# Autodesk Inventor assembly: RobotMK1
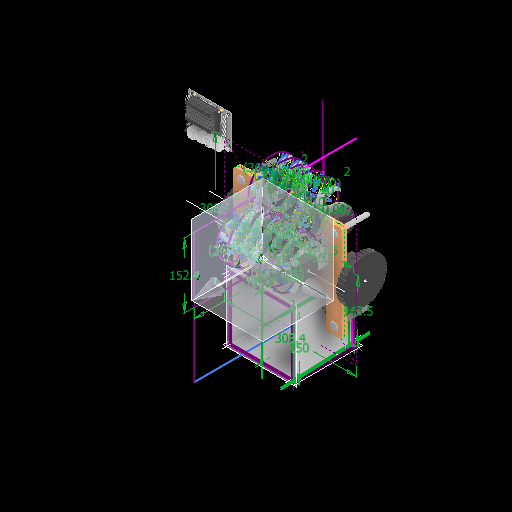
[picture p0: Inventor's stored thumbnail of the model, 512x512]
Saved by Autodesk Inventor 2025 (Build 290162000, 162)
## iProperties
Created: 2024-11-11
Part Number: RobotMK1
Document SubType Name: Assembly
Designer: Trevor
Author: Trevor
## Documents named in this file (18)
- C:\Users\Trevor\Documents\GitHub\USA-Robotic-Club-2024\assests\RobotMK1.iam
- C:\Users\Trevor\Documents\GitHub\USA-Robotic-Club-2024\assests\Newest base v1.ipt
- C:\Users\Trevor\Documents\GitHub\USA-Robotic-Club-2024\assests\17hm08-1204s-nema17-pancake-21mm-1.snapshot.2\17HM08-1204S Nema17 Pancake 21mm\17HM08-1204S Nema17 Pancake 21mm.ipt
- C:\Users\Trevor\Documents\GitHub\USA-Robotic-Club-2024\assests\Part147.ipt
- C:\Users\Trevor\Documents\GitHub\USA-Robotic-Club-2024\assests\nema-17-40mm-stepper-motor-1.snapshot.22\17HM15-0904S\17HM15-0904S\17HM15-0904S.ipt
- C:\Users\Trevor\Documents\GitHub\USA-Robotic-Club-2024\assests\RobotWheelMK1.ipt
- C:\Users\Trevor\Documents\GitHub\USA-Robotic-Club-2024\assests\Nema17WheelMotorMount.ipt
- C:\Users\Trevor\Documents\GitHub\USA-Robotic-Club-2024\assests\PancakeNema17MotorMount.ipt
- C:\Users\Trevor\Documents\GitHub\USA-Robotic-Club-2024\assests\DrivePillars.ipt
- C:\Users\Trevor\Documents\GitHub\USA-Robotic-Club-2024\assests\RodBearingMount.ipt
- C:\Users\Trevor\Documents\GitHub\USA-Robotic-Club-2024\assests\bearing-10mm-2.snapshot.2\PMG(Si)\PMG(Si).ipt
- C:\Users\Trevor\Documents\GitHub\USA-Robotic-Club-2024\assests\CombineRodSpace.ipt
- C:\Users\Trevor\Documents\GitHub\USA-Robotic-Club-2024\assests\Combine mk5.ipt
- C:\Users\Trevor\Documents\GitHub\USA-Robotic-Club-2024\assests\RodMK2.ipt
- C:\Users\Trevor\Documents\GitHub\USA-Robotic-Club-2024\assests\Bucket no fillets 2.ipt
- C:\Users\Trevor\Documents\GitHub\USA-Robotic-Club-2024\assests\nvidia-jetson-nano-2.snapshot.10\Jetson nano_fixed\Jetson nano_fixed.ipt
- C:\Users\Trevor\Documents\GitHub\USA-Robotic-Club-2024\assests\Layer2RodHolder.ipt
- C:\Users\Trevor\Documents\GitHub\USA-Robotic-Club-2024\assests\PancakeTopMount.ipt
## Components (41 placed, 17 different names)
1. Newest base v1:1 — Mate:9, Angle:1, Mate:10, Angle:2, Mate:22, Flush:1, Mate:23, Flush:2, Mate:28, Flush:3, Flush:4, Flush:6, Flush:8, Flush:9, Mate:51, Mate:52, Mate:53, Mate:54, Mate:55, Mate:56, Flush:10, Flush:12, Mate:88, Mate:89, Flush:13, Mate:90, Mate:91, Angle:3, Flush:21, Flush:22, Mate:101, Flush:24
2. 17HM15-0904S:1 — Mate:23, Flush:2, Mate:24, Mate:35, Mate:36, Mate:37, Mate:41, Mate:42
3. 17HM15-0904S:2 — Mate:22, Flush:1, Mate:25, Mate:32, Mate:33, Flush:5
4. 17HM08-1204S Nema17 Pancake 21mm:1 — Mate:28, Flush:3, Flush:4, Mate:29, Flush:7, Mate:57, Mate:58, Mate:65
5. RobotWheelMK1:1 — Mate:32, Mate:33, Mate:34
6. RobotWheelMK1:2 — Mate:35, Mate:36, Mate:38
7. Nema17WheelMotorMount:1 — Flush:5, Flush:6
8. Nema17WheelMotorMount:2 — Mate:41, Mate:42
9. PancakeNema17MotorMount:1 — Flush:7, Flush:8
10. DrivePillars:1 — Flush:9
11. DrivePillars:2 — Mate:51, Mate:55
12. DrivePillars:3 — Mate:52, Mate:56, Tangent:1
13. DrivePillars:4 — Mate:53, Mate:54
14. Part147:1 — Mate:57, Mate:58, Mate:63, Mate:64, Mate:66, Mate:68, Mate:70, Mate:72, Mate:74, Mate:76, Mate:78, Mate:80, Mate:82, Mate:84, Mate:86, Flush:14
15. PMG(Si):1 — Mate:63, Flush:10, Flush:11
16. RodBearingMount:1 — Flush:11, Flush:12
17. CombineRodSpace:1 — Mate:64, Mate:65, Mate:67, Flush:15
18. Combine mk5:1 — Mate:66, Mate:67, Mate:69
19. CombineRodSpace:3 — Mate:84, Mate:85, Mate:87, Flush:20
20. CombineRodSpace:4 — Mate:76, Mate:77, Mate:79, Flush:18
21. CombineRodSpace:5 — Mate:80, Mate:81, Mate:83, Flush:19
22. CombineRodSpace:7 — Mate:72, Mate:73, Mate:75, Flush:17
23. CombineRodSpace:8 — Mate:68, Mate:69, Mate:71, Flush:16
24. Combine mk5:2 — Mate:82, Mate:83, Mate:85
25. Combine mk5:3 — Mate:78, Mate:79, Mate:81
26. Combine mk5:4 — Mate:74, Mate:75, Mate:77
27. Combine mk5:5 — Mate:70, Mate:71, Mate:73
28. Combine mk5:6 — Mate:86, Mate:87
29. RodMK2:1 — Mate:90, Flush:14, Mate:92, Mate:93, Mate:94, Mate:95, Mate:96, Mate:97, Mate:98, Mate:100
30. 17HM08-1204S Nema17 Pancake 21mm:2 — Mate:91, Mate:92, Flush:23
31. Combine mk5:7 — Mate:97, Flush:19
32. Combine mk5:8 — Mate:95, Flush:17
33. Combine mk5:9 — Mate:93, Flush:15
34. Combine mk5:10 — Mate:96, Flush:18
35. Combine mk5:11 — Mate:94, Flush:16
36. Combine mk5:12 — Mate:98, Flush:20
37. Bucket no fillets 2:1 — Mate:99
38. Jetson nano_fixed:1
39. Layer2RodHolder:1 — Flush:21, Flush:22
40. PMG(Si):2 — Mate:100, Mate:101
41. PancakeTopMount:1 — Flush:23, Flush:24
## Relationships (98: Mate 69, Flush 24, Angle 3, Symmetry 1, Tangent 1)
- Mate:8
- Mate:9: Newest base v1:1
- Angle:1 (0 deg): Newest base v1:1
- Mate:10: Newest base v1:1
- Angle:2 (0 deg): Newest base v1:1
- Symmetry:1
- Mate:21
- Mate:22: Newest base v1:1 ↔ 17HM15-0904S:2
- Flush:1: Newest base v1:1 ↔ 17HM15-0904S:2
- Mate:23: Newest base v1:1 ↔ 17HM15-0904S:1
- Flush:2: Newest base v1:1 ↔ 17HM15-0904S:1
- Mate:24: 17HM15-0904S:1
- Mate:25: 17HM15-0904S:2
- Mate:26
- Mate:27
- Mate:28: Newest base v1:1 ↔ 17HM08-1204S Nema17 Pancake 21mm:1
- Flush:3: Newest base v1:1 ↔ 17HM08-1204S Nema17 Pancake 21mm:1
- Flush:4: Newest base v1:1 ↔ 17HM08-1204S Nema17 Pancake 21mm:1
- Mate:29: 17HM08-1204S Nema17 Pancake 21mm:1
- Mate:30
- Mate:32: 17HM15-0904S:2 ↔ RobotWheelMK1:1
- Mate:33: 17HM15-0904S:2 ↔ RobotWheelMK1:1
- Mate:34: RobotWheelMK1:1
- Mate:35: 17HM15-0904S:1 ↔ RobotWheelMK1:2
- Mate:36: 17HM15-0904S:1 ↔ RobotWheelMK1:2
- Mate:37: 17HM15-0904S:1
- Mate:38: RobotWheelMK1:2
- Flush:5: 17HM15-0904S:2 ↔ Nema17WheelMotorMount:1
- Flush:6: Newest base v1:1 ↔ Nema17WheelMotorMount:1
- Mate:41: 17HM15-0904S:1 ↔ Nema17WheelMotorMount:2
- Mate:42: 17HM15-0904S:1 ↔ Nema17WheelMotorMount:2
- Flush:7: 17HM08-1204S Nema17 Pancake 21mm:1 ↔ PancakeNema17MotorMount:1
- Flush:8: Newest base v1:1 ↔ PancakeNema17MotorMount:1
- Flush:9: Newest base v1:1 ↔ DrivePillars:1
- Mate:51: Newest base v1:1 ↔ DrivePillars:2
- Mate:52: Newest base v1:1 ↔ DrivePillars:3
- Mate:53: Newest base v1:1 ↔ DrivePillars:4
- Mate:54: Newest base v1:1 ↔ DrivePillars:4
- Mate:55: Newest base v1:1 ↔ DrivePillars:2
- Mate:56: Newest base v1:1 ↔ DrivePillars:3
- Mate:57: 17HM08-1204S Nema17 Pancake 21mm:1 ↔ Part147:1
- Mate:58: 17HM08-1204S Nema17 Pancake 21mm:1 ↔ Part147:1
- Mate:63: Part147:1 ↔ PMG(Si):1
- Flush:10: Newest base v1:1 ↔ PMG(Si):1
- Flush:11: PMG(Si):1 ↔ RodBearingMount:1
- Flush:12: Newest base v1:1 ↔ RodBearingMount:1
- Mate:64: Part147:1 ↔ CombineRodSpace:1
- Mate:65: 17HM08-1204S Nema17 Pancake 21mm:1 ↔ CombineRodSpace:1
- Mate:66: Part147:1 ↔ Combine mk5:1
- Mate:67: CombineRodSpace:1 ↔ Combine mk5:1
- Mate:68: Part147:1 ↔ CombineRodSpace:8
- Mate:69: Combine mk5:1 ↔ CombineRodSpace:8
- Mate:70: Part147:1 ↔ Combine mk5:5
- Mate:71: CombineRodSpace:8 ↔ Combine mk5:5
- Mate:72: Part147:1 ↔ CombineRodSpace:7
- Mate:73: CombineRodSpace:7 ↔ Combine mk5:5
- Mate:74: Part147:1 ↔ Combine mk5:4
- Mate:75: CombineRodSpace:7 ↔ Combine mk5:4
- Mate:76: Part147:1 ↔ CombineRodSpace:4
- Mate:77: CombineRodSpace:4 ↔ Combine mk5:4
- Mate:78: Part147:1 ↔ Combine mk5:3
- Mate:79: CombineRodSpace:4 ↔ Combine mk5:3
- Mate:80: Part147:1 ↔ CombineRodSpace:5
- Mate:81: CombineRodSpace:5 ↔ Combine mk5:3
- Mate:82: Part147:1 ↔ Combine mk5:2
- Mate:83: CombineRodSpace:5 ↔ Combine mk5:2
- Mate:84: Part147:1 ↔ CombineRodSpace:3
- Mate:85: CombineRodSpace:3 ↔ Combine mk5:2
- Mate:86: Part147:1 ↔ Combine mk5:6
- Mate:87: CombineRodSpace:3 ↔ Combine mk5:6
- Mate:88: Newest base v1:1
- Mate:89: Newest base v1:1
- Flush:13: Newest base v1:1
- Mate:90: Newest base v1:1 ↔ RodMK2:1
- Flush:14: Part147:1 ↔ RodMK2:1
- Mate:91: Newest base v1:1 ↔ 17HM08-1204S Nema17 Pancake 21mm:2
- Mate:92: RodMK2:1 ↔ 17HM08-1204S Nema17 Pancake 21mm:2
- Mate:93: RodMK2:1 ↔ Combine mk5:9
- Flush:15: CombineRodSpace:1 ↔ Combine mk5:9
- Mate:94: RodMK2:1 ↔ Combine mk5:11
- Flush:16: CombineRodSpace:8 ↔ Combine mk5:11
- Mate:95: RodMK2:1 ↔ Combine mk5:8
- Flush:17: CombineRodSpace:7 ↔ Combine mk5:8
- Mate:96: RodMK2:1 ↔ Combine mk5:10
- Flush:18: CombineRodSpace:4 ↔ Combine mk5:10
- Mate:97: RodMK2:1 ↔ Combine mk5:7
- Flush:19: CombineRodSpace:5 ↔ Combine mk5:7
- Mate:98: RodMK2:1 ↔ Combine mk5:12
- Flush:20: CombineRodSpace:3 ↔ Combine mk5:12
- Angle:3 (0 deg): Newest base v1:1
- Tangent:1: DrivePillars:3
- Mate:99: Bucket no fillets 2:1
- Flush:21: Newest base v1:1 ↔ Layer2RodHolder:1
- Flush:22: Newest base v1:1 ↔ Layer2RodHolder:1
- Mate:100: RodMK2:1 ↔ PMG(Si):2
- Mate:101: Newest base v1:1 ↔ PMG(Si):2
- Flush:23: 17HM08-1204S Nema17 Pancake 21mm:2 ↔ PancakeTopMount:1
- Flush:24: Newest base v1:1 ↔ PancakeTopMount:1
